# Autodesk Inventor assembly: Top Arm-N
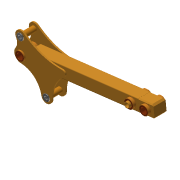
[picture p0: Inventor's stored thumbnail of the model, 180x180]
Saved by Autodesk Inventor 2022 Beta2 (Build 260130000, 130) ContinuousBuild 0
## iProperties
Shininess: 64.0
Length Units: 11269
Angle Units: 11279
Time Units: 11290
Mass Units: 11283
Length Display Precision: 3
Angle Display Precision: 2
Compacted: True
Created: 2003-04-13
Part Number: Top Arm-N
Document SubType Name: Assembly
Designer: Uffe Bak
Density: 0.0
Volumn: 0.0
Area: 0.0
PropertySet Name: Model Information
Control State: 0
Master: False
Checked Out: False
Author: Uffe Bak
## Documents named in this file (6)
- C:\Autodesk Inventor 2021 Intro Practice Files\BOM\Top Arm-N.iam
- C:\Autodesk Inventor 2021 Intro Practice Files\BOM\3136 1133 84.iam
- C:\Autodesk Inventor 2021 Intro Practice Files\BOM\3136 7044 74.ipt
- C:\Autodesk Inventor 2021 Intro Practice Files\BOM\3136 7044 79.ipt
- C:\Autodesk Inventor 2021 Intro Practice Files\BOM\3136 7057 14.ipt
- C:\Autodesk Inventor 2021 Intro Practice Files\BOM\3136 7044 91.ipt
## Components (12 placed, 5 different names)
1. 3136 1133 84:1 [sub-assembly] — Insert:1, Insert:2, Insert:10
2. 3136 7044 74:1 — Insert:1, Insert:3, Insert:6
3. 3136 7044 79:1 — Insert:3, Insert:27
4. 3136 7057 14:1 — Insert:27
5. 3136 7044 91:1 — Insert:10
6. 3136 7044 74:2 — Insert:2, Insert:4, Insert:8
7. 3136 7044 79:2 — Insert:6, Insert:7
8. 3136 7044 79:3 — Insert:4, Insert:5
9. 3136 7044 79:4 — Insert:8, Insert:9
10. 3136 7057 14:2 — Insert:7
11. 3136 7057 14:3 — Insert:5
12. 3136 7057 14:4 — Insert:9
## Relationships (11: Insert 11)
- Insert:1 (2.25 mm): 3136 1133 84:1 ↔ 3136 7044 74:1
- Insert:2 (2.25 mm): 3136 1133 84:1 ↔ 3136 7044 74:2
- Insert:3: 3136 7044 74:1 ↔ 3136 7044 79:1
- Insert:4: 3136 7044 74:2 ↔ 3136 7044 79:3
- Insert:5: 3136 7044 79:3 ↔ 3136 7057 14:3
- Insert:6: 3136 7044 74:1 ↔ 3136 7044 79:2
- Insert:7: 3136 7044 79:2 ↔ 3136 7057 14:2
- Insert:8: 3136 7044 74:2 ↔ 3136 7044 79:4
- Insert:9: 3136 7044 79:4 ↔ 3136 7057 14:4
- Insert:10 (12.25 mm): 3136 1133 84:1 ↔ 3136 7044 91:1
- Insert:27: 3136 7044 79:1 ↔ 3136 7057 14:1
